# Autodesk Inventor assembly: Vented plug
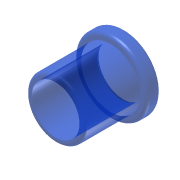
[picture p0: Inventor's stored thumbnail of the model, 180x180]
Saved by Autodesk Inventor 2014 (Build 180170000, 170)
## iProperties
Created: 2016-08-28
Part Number: Vented plug
Document SubType Name: Assembly
Designer: Camilo
Author: Camilo
## Documents named in this file (2)
- Z:\Github\AgingTests\3D parts\Vented plug\Vented plug.iam
- Z:\Github\AgingTests\3D parts\ECoG holder\flaskPort.ipt
## Components (1 placed, 1 different names)
1. flaskPort:1 — Mate:1, Flush:1, Mate:2
## Relationships (3: Mate 2, Flush 1)
- Mate:1: flaskPort:1
- Flush:1: flaskPort:1
- Mate:2: flaskPort:1
